# Autodesk Inventor assembly: Estante3
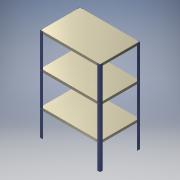
[picture p0: Inventor's stored thumbnail of the model, 180x180]
Saved by Autodesk Inventor 2016 (Build 200138000, 138)
## iProperties
Created: 2015-11-12
Part Number: Estante3
Material: Genérico
Document SubType Name: Assembly
Designer: David
_SolveAssemblyDoc: Frame Generator Solve Assembly
_Version: 15.0.0
Author: David
## Documents named in this file (5)
- D:\mis documentos\david\computaciuon grafica\proyecto final\mod\Proyecto computación Gráfica\Cuarto Refrigerante\Cuerpo Principal\Modelado\estantería\estantería\Estante3.iam
- D:\mis documentos\david\computaciuon grafica\proyecto final\mod\Proyecto computación Gráfica\Cuarto Refrigerante\Cuerpo Principal\Modelado\estantería\estantería\Esqueleto.ipt
- D:\mis documentos\david\computaciuon grafica\proyecto final\mod\Proyecto computación Gráfica\Cuarto Refrigerante\Cuerpo Principal\Modelado\estantería\estantería\Estante\Frame\Frame0001.iam
- D:\mis documentos\david\computaciuon grafica\proyecto final\mod\Proyecto computación Gráfica\Cuarto Refrigerante\Cuerpo Principal\Modelado\estantería\estantería\lámina.ipt
- D:\mis documentos\david\computaciuon grafica\proyecto final\mod\Proyecto computación Gráfica\Cuarto Refrigerante\Cuerpo Principal\Modelado\estantería\estantería\HBOLT 0.2500-20x1x0.75-S.ipt
## Components (17 placed, 4 different names)
1. Esqueleto:1
2. Frame0001:1 [sub-assembly] — Coincidencia:1, Coincidencia:2, Coincidencia:4, Coincidencia:10, Coincidencia:12, Coincidencia:14, Coincidencia:20, Coincidencia:22, Coincidencia:23, Coincidencia:30, Coincidencia:32, Coincidencia:33
3. lámina:2 — Nivelación:12, Nivelación:13
4. lámina:3 — Nivelación:8, Nivelación:9, Nivelación:10
5. lámina:4 — Nivelación:8, Nivelación:9, Nivelación:10, Nivelación:12, Nivelación:13
6. HBOLT 0.2500-20x1x0.75-S:1 — Coincidencia:1
7. HBOLT 0.2500-20x1x0.75-S:2 — Coincidencia:10
8. HBOLT 0.2500-20x1x0.75-S:3 — Coincidencia:2
9. HBOLT 0.2500-20x1x0.75-S:6 — Coincidencia:12
10. HBOLT 0.2500-20x1x0.75-S:7 — Coincidencia:4
11. HBOLT 0.2500-20x1x0.75-S:10 — Coincidencia:14
12. HBOLT 0.2500-20x1x0.75-S:11 — Coincidencia:20
13. HBOLT 0.2500-20x1x0.75-S:12 — Coincidencia:22
14. HBOLT 0.2500-20x1x0.75-S:13 — Coincidencia:32
15. HBOLT 0.2500-20x1x0.75-S:17 — Coincidencia:30
16. HBOLT 0.2500-20x1x0.75-S:19 — Coincidencia:33
17. HBOLT 0.2500-20x1x0.75-S:20 — Coincidencia:23
## Relationships (17: Mate 12, Flush 5)
- Nivelación:8 [Flush] (500 mm): lámina:3 ↔ lámina:4
- Nivelación:9 [Flush]: lámina:3 ↔ lámina:4
- Nivelación:10 [Flush]: lámina:3 ↔ lámina:4
- Nivelación:12 [Flush] (500 mm): lámina:2 ↔ lámina:4
- Nivelación:13 [Flush]: lámina:2 ↔ lámina:4
- Coincidencia:1 [Mate]: Frame0001:1 ↔ HBOLT 0.2500-20x1x0.75-S:1
- Coincidencia:2 [Mate]: Frame0001:1 ↔ HBOLT 0.2500-20x1x0.75-S:3
- Coincidencia:4 [Mate]: Frame0001:1 ↔ HBOLT 0.2500-20x1x0.75-S:7
- Coincidencia:10 [Mate]: Frame0001:1 ↔ HBOLT 0.2500-20x1x0.75-S:2
- Coincidencia:12 [Mate]: Frame0001:1 ↔ HBOLT 0.2500-20x1x0.75-S:6
- Coincidencia:14 [Mate]: Frame0001:1 ↔ HBOLT 0.2500-20x1x0.75-S:10
- Coincidencia:20 [Mate]: Frame0001:1 ↔ HBOLT 0.2500-20x1x0.75-S:11
- Coincidencia:22 [Mate]: Frame0001:1 ↔ HBOLT 0.2500-20x1x0.75-S:12
- Coincidencia:23 [Mate]: Frame0001:1 ↔ HBOLT 0.2500-20x1x0.75-S:20
- Coincidencia:30 [Mate]: Frame0001:1 ↔ HBOLT 0.2500-20x1x0.75-S:17
- Coincidencia:32 [Mate]: Frame0001:1 ↔ HBOLT 0.2500-20x1x0.75-S:13
- Coincidencia:33 [Mate]: Frame0001:1 ↔ HBOLT 0.2500-20x1x0.75-S:19
